# Autodesk Inventor assembly: BD Gearbox and Bracket Assy 2
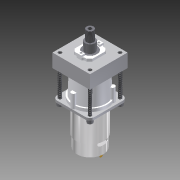
[picture p0: Inventor's stored thumbnail of the model, 180x180]
Saved by Autodesk Inventor 2012 (Build 160160000, 160)
## iProperties
Created: 2012-07-05
Part Number: BD Gearbox and Bracket Assy 2
Document SubType Name: Assembly
Designer: Bruce
Author: Bruce
## Documents named in this file (5)
- C:\Household Files\Bruce Work\Inventor Projects\2012 Swerve Drive\BD Drill Motor Gearbox\BD Gearbox and Bracket Assy 2.iam
- C:\Household Files\Bruce Work\Inventor Projects\2012 Swerve Drive\BD Drill Motor Gearbox\BD gearbox mount block.ipt
- C:\Household Files\Bruce Work\Inventor Projects\2012 Swerve Drive\BD Drill Motor Gearbox\BD Drill motor assembly.iam
- C:\Household Files\Bruce Work\Inventor Projects\2012 Swerve Drive\BD Drill Motor Gearbox\BD gearbox mount block motor ring.ipt
- C:\Household Files\Bruce Work\Inventor Projects\2012 Swerve Drive\BD Drill Motor Gearbox\Bolt 8-32 bracket BD Drill motor mount.ipt
## Components (7 placed, 4 different names)
1. BD gearbox mount block:1 — Mate:1, Mate:2, Mate:3, Mate:4, Mate:6
2. BD Drill motor assembly:1 [sub-assembly] — Mate:1, Mate:2, Mate:3, Mate:5
3. BD gearbox mount block motor ring:1 — Mate:4, Mate:5, Mate:6, Mate:7, Mate:8, Insert:1, Insert:2, Insert:3
4. Bolt 8-32 bracket BD Drill motor mount:1 — Mate:7, Mate:8
5. Bolt 8-32 bracket BD Drill motor mount:2 — Insert:3
6. Bolt 8-32 bracket BD Drill motor mount:3 — Insert:2
7. Bolt 8-32 bracket BD Drill motor mount:4 — Insert:1
## Relationships (11: Mate 8, Insert 3)
- Mate:1: BD gearbox mount block:1 ↔ BD Drill motor assembly:1
- Mate:2: BD gearbox mount block:1 ↔ BD Drill motor assembly:1
- Mate:3: BD gearbox mount block:1 ↔ BD Drill motor assembly:1
- Mate:4: BD gearbox mount block:1 ↔ BD gearbox mount block motor ring:1
- Mate:5: BD Drill motor assembly:1 ↔ BD gearbox mount block motor ring:1
- Mate:6: BD gearbox mount block:1 ↔ BD gearbox mount block motor ring:1
- Mate:7: BD gearbox mount block motor ring:1 ↔ Bolt 8-32 bracket BD Drill motor mount:1
- Mate:8: BD gearbox mount block motor ring:1 ↔ Bolt 8-32 bracket BD Drill motor mount:1
- Insert:1: BD gearbox mount block motor ring:1 ↔ Bolt 8-32 bracket BD Drill motor mount:4
- Insert:2: BD gearbox mount block motor ring:1 ↔ Bolt 8-32 bracket BD Drill motor mount:3
- Insert:3: BD gearbox mount block motor ring:1 ↔ Bolt 8-32 bracket BD Drill motor mount:2
